# Autodesk Inventor assembly: hpr station TOPLEVEL
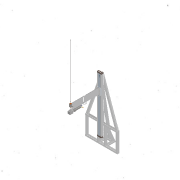
[picture p0: Inventor's stored thumbnail of the model, 180x180]
Saved by Autodesk Inventor 2021 (Build 250183000, 183)
## iProperties
Created: 2021-03-29
Part Number: hpr station TOPLEVEL
Document SubType Name: Assembly
Designer: Work
Author: Work
## Documents named in this file (11)
- C:\Users\Work\OneDrive - Brookhaven National Laboratory\Daniels, William intern HPR station\hpr station TOPLEVEL.iam
- C:\Users\Work\OneDrive - Brookhaven National Laboratory\Daniels, William intern HPR station\Actuator\CKK_145_NN_1_1800_mm_MF01_03_34_309_033.iam
- C:\Users\Work\OneDrive - Brookhaven National Laboratory\Daniels, William intern HPR station\Arm\arm TOPLEVEL.iam
- C:\Users\Work\OneDrive - Brookhaven National Laboratory\Daniels, William intern HPR station\Frame\frame TOPLEVEL.iam
- C:\Users\Work\OneDrive - Brookhaven National Laboratory\Daniels, William intern HPR station\hpr station TOPLEVEL\AIP\FEA\dk6q0yb6o.fins
- C:\Users\Work\OneDrive - Brookhaven National Laboratory\Daniels, William intern HPR station\hpr station TOPLEVEL\AIP\FEA\dk6q0yb6o.fsat
- C:\Users\Work\OneDrive - Brookhaven National Laboratory\Daniels, William intern HPR station\hpr station TOPLEVEL\AIP\FEA\dk6q0yb6o.ftes
- C:\Users\Work\OneDrive - Brookhaven National Laboratory\Daniels, William intern HPR station\hpr station TOPLEVEL\AIP\FEA\dk6q0yb7k.fwiz
- C:\Users\Work\OneDrive - Brookhaven National Laboratory\Daniels, William intern HPR station\hpr station TOPLEVEL\AIP\FEA\dk6q0ybnk.fmsh
- C:\Users\Work\OneDrive - Brookhaven National Laboratory\Daniels, William intern HPR station\hpr station TOPLEVEL\AIP\FEA\dk6q0ybnl.fres
- C:\Users\Work\OneDrive - Brookhaven National Laboratory\Daniels, William intern HPR station\dimensions.xlsx
## Components (3 placed, 3 different names)
1. CKK_145_NN_1_1800_mm_MF01_03_34_309_033:1 [sub-assembly] — Rigid:1, Rigid:2
2. arm TOPLEVEL:1 [sub-assembly] — Rigid:1
3. frame TOPLEVEL:1 [sub-assembly] — Rigid:2
## Relationships (2: WeldJoint 2)
- Rigid:1 [WeldJoint]: CKK_145_NN_1_1800_mm_MF01_03_34_309_033:1 ↔ arm TOPLEVEL:1
- Rigid:2 [WeldJoint] (0.008 mm): CKK_145_NN_1_1800_mm_MF01_03_34_309_033:1 ↔ frame TOPLEVEL:1
## Named parameters: sa_0 = 980.999, height = 203.2 mm, thickness = 12.7 mm, shaftDiam = 6.35 mm, shaftSpace = 1.5875 mm, stageSpace = 2.54 mm, stageAngle = 15 deg, bearingDiam = 9.5504 mm, FlangeDiam = 12.7 mm, FlangeDepth = 1.5875 mm, smallFilet = 0.39687 mm, ringDiam = 96.46608 mm, stockHeight = 50.8 mm, stockWidth = 76.2 mm, stockRad = 9.525 mm, stockGuage = 3.175 mm, actuHieght = 1800 mm, groundActu = 304.8 mm, baseWidth = 1066.8 mm, baseDepth = 254 mm, capThickness = 3.175 mm, sup1Len = 660.4 mm, sup1Ang = 22.619865 deg, sup2Len = 2079.37366 mm, sup2Ang = 8.959949 deg, supVertLen = 955.13561 mm, supSideLen = 1531.12879 mm, supSideAng = 19.376933 deg
note: some values were not read from the file. Shown as the stored number, unit unknown: "sa_0".
